# Autodesk Inventor assembly: mag_6mm
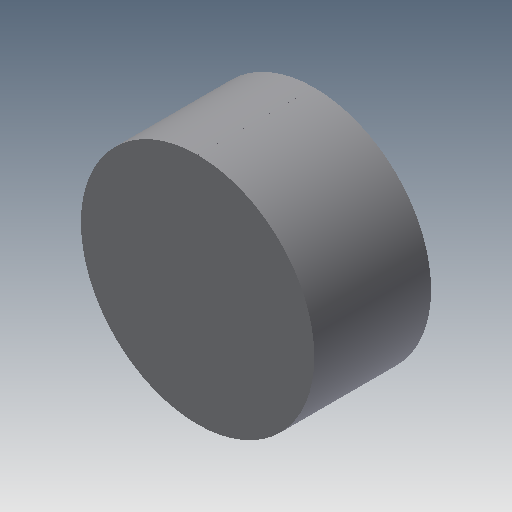
[picture p0: Inventor's stored thumbnail of the model, 512x512]
Saved by Autodesk Inventor 2020.3 (Build 243373000, 373)
## iProperties
Created: 2020-11-15
Part Number: mag_6mm
Document SubType Name: Assembly
Designer: paulg
Author: paulg
## Documents named in this file (2)
- F:\UQ Engineering\2021 ~ 5th Year\Semester 2\METR4911-THESIS\FarmBot CAD\FarmBotV1\CycloidalJoint\Cycloid CAD\mag_6mm.iam
- F:\UQ Engineering\2021 ~ 5th Year\Semester 2\METR4911-THESIS\FarmBot CAD\FarmBotV1\CycloidalJoint\Cycloid CAD\half_mag.ipt
## Components (2 placed, 1 different names)
1. half_mag:1 — Mate:1, Flush:1, Insert:1
2. half_mag:2 — Mate:1, Flush:1, Insert:1
## Relationships (3: Mate 1, Flush 1, Insert 1)
- Mate:1: half_mag:1 ↔ half_mag:2
- Flush:1: half_mag:1 ↔ half_mag:2
- Insert:1: half_mag:1 ↔ half_mag:2
